# Autodesk Inventor assembly: testAssambly
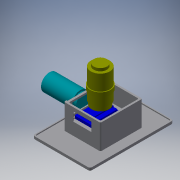
[picture p0: Inventor's stored thumbnail of the model, 180x180]
Saved by Autodesk Inventor 2016 (Build 200138000, 138)
## iProperties
Created: 2016-11-02
Part Number: testAssambly
Document SubType Name: Assembly
Designer: sims01
Author: sims01
## Documents named in this file (6)
- H:\Documents\LSFM_3\setup\mechanical\design\sampleHolderDesign\testAssambly.iam
- H:\Documents\LSFM_3\setup\mechanical\design\sampleHolderDesign\sampleChamberExt.ipt
- H:\Documents\LSFM_3\setup\mechanical\design\lsfm3_mechDesign\olympusXLSLPLN25XGMP_vFIN.ipt
- H:\Documents\LSFM_3\setup\mechanical\design\lsfm3_mechDesign\10X_mitutoyoObj.ipt
- H:\Documents\LSFM_3\setup\mechanical\design\sampleHolderDesign\sampleChamberInterior.ipt
- H:\Documents\LSFM_3\setup\mechanical\design\sampleHolderDesign\sampleChamberExt_v1.ipt
## Components (5 placed, 5 different names)
1. sampleChamberExt:1
2. olympusXLSLPLN25XGMP_vFIN:1 — Mate:1, Mate:2, Mate:3
3. 10X_mitutoyoObj:1 — Mate:4, Mate:5, Mate:6
4. sampleChamberInterior:1 — Flush:1, Rigid:1
5. sampleChamberExt_v1:1 — Rigid:1
## Relationships (8: Mate 6, Flush 1, WeldJoint 1)
- Mate:1: olympusXLSLPLN25XGMP_vFIN:1
- Mate:2 (8 mm): olympusXLSLPLN25XGMP_vFIN:1
- Mate:3: olympusXLSLPLN25XGMP_vFIN:1
- Mate:4: 10X_mitutoyoObj:1
- Mate:5: 10X_mitutoyoObj:1
- Mate:6 (-33 mm): 10X_mitutoyoObj:1
- Flush:1: sampleChamberInterior:1
- Rigid:1 [WeldJoint]: sampleChamberInterior:1 ↔ sampleChamberExt_v1:1
